# Autodesk Inventor assembly: Skrzydlo sterowe_MIR
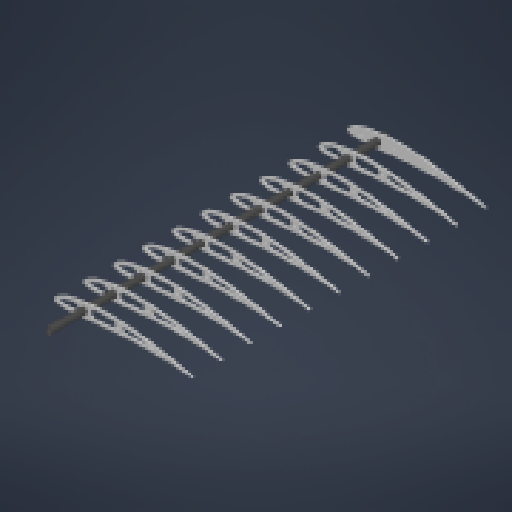
[picture p0: Inventor's stored thumbnail of the model, 512x512]
Saved by Autodesk Inventor 2023 (Build 270158000, 158)
## iProperties
Created: 2022-12-09
Part Number: Skrzydlo sterowe_MIR
Document SubType Name: Assembly
Designer: szykr
Author: szykr
## Documents named in this file (6)
- D:\Folder Instalacyjny\GitHub Pliki\Solaris\model\Skrzydlo sterowe_MIR.iam
- D:\Folder Instalacyjny\GitHub Pliki\Solaris\model\Wingspar trochemniejnizpol metrowy_MIR.ipt
- D:\Folder Instalacyjny\GitHub Pliki\Solaris\model\Żebro Montaż_MIR.ipt
- D:\Folder Instalacyjny\GitHub Pliki\Solaris\model\Żebro Default_MIR.ipt
- D:\Folder Instalacyjny\GitHub Pliki\Solaris\model\Zebro_lotka_serwo_MIR.iam
- D:\Folder Instalacyjny\GitHub Pliki\Solaris\model\Zebro_lotka_normal_MIR.iam
## Components (12 placed, 5 different names)
1. Wingspar trochemniejnizpol metrowy_MIR:1 — Insert:1
2. Żebro Montaż_MIR:1 — Insert:1, Angle:1, Insert:5, Insert:3, Insert:2
3. Zebro_lotka_serwo_MIR:1 [sub-assembly] — Insert:4, Insert:3
4. Żebro Default_MIR:2 — Insert:5
5. Żebro Default_MIR:3
6. Zebro_lotka_normal_MIR:1 [sub-assembly] — Insert:4
7. Zebro_lotka_normal_MIR:2 [sub-assembly]
8. Zebro_lotka_normal_MIR:3 [sub-assembly]
9. Zebro_lotka_normal_MIR:4 [sub-assembly]
10. Zebro_lotka_normal_MIR:5 [sub-assembly]
11. Żebro Default_MIR:1 — Insert:2
12. Żebro Default_MIR:4
## Component patterns: (2 elements, first: Żebro Default_MIR:2), (5 elements, first: Zebro_lotka_normal_MIR:1), (2 elements, first: Żebro Default_MIR:1)
## Relationships (6: Insert 5, Angle 1)
- Insert:1 (9 mm): Wingspar trochemniejnizpol metrowy_MIR:1 ↔ Żebro Montaż_MIR:1
- Angle:1 (90 deg): Żebro Montaż_MIR:1
- Insert:5 (382.091 mm): Żebro Montaż_MIR:1 ↔ Żebro Default_MIR:2
- Insert:4 (42.455 mm): Zebro_lotka_serwo_MIR:1 ↔ Zebro_lotka_normal_MIR:1
- Insert:3 (127.364 mm): Żebro Montaż_MIR:1 ↔ Zebro_lotka_serwo_MIR:1
- Insert:2 (42.455 mm): Żebro Montaż_MIR:1 ↔ Żebro Default_MIR:1
## Named parameters: ilosc_zeber_przed = 2, ilosc_lotek = 5, ilosc_zeber_po = 2, ilosc_zeber_full = 11, length_wingspara = 488 mm, length_true = 467 mm, spacing = 42.455 mm
